# Autodesk Inventor assembly: skellett
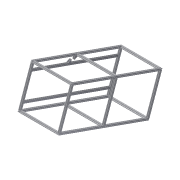
[picture p0: Inventor's stored thumbnail of the model, 180x180]
Saved by Autodesk Inventor 2014 SP1 (Build 180222100, 222)
## iProperties
Created: 2015-02-04
Part Number: skellett
Document SubType Name: Assembly
Designer: Simen
Author: Simen
## Documents named in this file (9)
- C:\Users\Simen\Documents\git\Eit\skjellet\skellett.iam
- C:\Users\Simen\Documents\git\Eit\skjellet\KHFS5_2020_1000.ipt
- C:\Users\Simen\Documents\git\Eit\skjellet\KHFS5_2020_486.ipt
- C:\Users\Simen\Documents\git\Eit\skjellet\KHFS5_2020_386.ipt
- C:\Users\Simen\Documents\git\Eit\skjellet\KHFS5_2020_381.ipt
- C:\Users\Simen\Documents\git\Eit\skjellet\KHFS5_2020_391.ipt
- C:\Users\Simen\Documents\git\Eit\skjellet\KHFS5_2020_960.ipt
- C:\Users\Simen\Documents\git\Eit\skjellet\KHFS5_2020_47.ipt
- C:\Users\Simen\Documents\git\Eit\skjellet\jorneFester.iam
## Components (26 placed, 2 different names)
1. KHFS5-2020-4000:12 — Mate:44, Flush:60, Flush:61, Flush:62, Flush:63, Mate:45, Mate:46, Mate:47, Flush:64, Flush:65, Flush:66, Flush:77, Flush:78, Mate:59
2. KHFS5-2020-4000:13 — Mate:36, Mate:37, Flush:45, Flush:46, Flush:47, Flush:48, Mate:39, Flush:56, Flush:57, Mate:52, Flush:71, Mate:62, Flush:81, Flush:82, Mate:67, Flush:88, Flush:89
3. KHFS5-2020-4000:14 — Mate:33, Mate:34, Mate:35, Flush:42, Flush:43, Flush:44, Flush:49, Flush:50, Flush:51, Mate:38, Mate:40, Mate:41, Flush:52, Flush:53, Flush:54, Flush:55, Flush:80, Mate:65, Flush:83, Mate:66, Flush:85, Flush:86, Flush:87
4. KHFS5-2020-4000:15 — Mate:43, Flush:58, Flush:59, Mate:53, Flush:73, Flush:75, Mate:56, Flush:76, Mate:58
5. KHFS5-2020-4000:25 — Mate:33, Flush:44, Flush:49
6. KHFS5-2020-4000:26 — Mate:34, Flush:43, Flush:51, Flush:67, Flush:68
7. KHFS5-2020-4000:27 — Mate:35, Flush:42, Flush:50, Flush:62, Flush:63, Mate:45
8. KHFS5-2020-4000:36 — Flush:69, Mate:50, Mate:55, Mate:58, Mate:63
9. KHFS5-2020-4000:28 — Mate:36, Flush:45, Flush:48, Flush:69, Mate:49, Flush:70
10. KHFS5-2020-4000:29 — Mate:37, Flush:46, Flush:47
11. KHFS5-2020-4000:30 — Mate:38, Mate:39, Flush:52, Flush:53, Flush:56, Flush:57
12. KHFS5-2020-4000:31 — Mate:40, Flush:54, Flush:68, Flush:72, Flush:84
13. KHFS5-2020-4000:32 — Mate:43, Flush:58, Flush:59, Mate:44, Flush:60, Flush:61
14. KHFS5-2020-4000:33 — Mate:41, Flush:55, Flush:87
15. KHFS5-2020-4000:34 — Mate:47, Flush:64, Flush:66
16. KHFS5-2020-4000:42 — Mate:62, Flush:81, Flush:82, Mate:63, Mate:64
17. KHFS5-2020-4000:43 — Mate:65, Flush:83, Flush:84
18. KHFS5-2020-4000:35 — Mate:46, Flush:65, Flush:67, Flush:74
19. KHFS5-2020-4000:37 — Mate:49, Flush:70, Mate:50, Mate:64
20. KHFS5-2020-4000:40 — Flush:77, Flush:78, Mate:59, Flush:80
21. KHFS5-2020-4000:38 — Mate:52, Flush:71, Flush:72
22. KHFS5-2020-4000:39 — Mate:53, Flush:73, Flush:74, Mate:54, Mate:57
23. jorneFester:1 [sub-assembly] — Mate:56, Mate:57, Flush:76
24. jorneFester:2 [sub-assembly] — Mate:54, Flush:75, Mate:55
25. KHFS5-2020-4000:44 — Mate:66, Flush:85, Flush:86
26. KHFS5-2020-4000:45 — Mate:67, Flush:88, Flush:89
## Relationships (78: Flush 47, Mate 31)
- Mate:33: KHFS5-2020-4000:14 ↔ KHFS5-2020-4000:25
- Mate:34: KHFS5-2020-4000:14 ↔ KHFS5-2020-4000:26
- Mate:35: KHFS5-2020-4000:14 ↔ KHFS5-2020-4000:27
- Mate:36: KHFS5-2020-4000:13 ↔ KHFS5-2020-4000:28
- Mate:37: KHFS5-2020-4000:13 ↔ KHFS5-2020-4000:29
- Flush:42: KHFS5-2020-4000:14 ↔ KHFS5-2020-4000:27
- Flush:43: KHFS5-2020-4000:14 ↔ KHFS5-2020-4000:26
- Flush:44: KHFS5-2020-4000:14 ↔ KHFS5-2020-4000:25
- Flush:45: KHFS5-2020-4000:13 ↔ KHFS5-2020-4000:28
- Flush:46: KHFS5-2020-4000:13 ↔ KHFS5-2020-4000:29
- Flush:47: KHFS5-2020-4000:13 ↔ KHFS5-2020-4000:29
- Flush:48: KHFS5-2020-4000:13 ↔ KHFS5-2020-4000:28
- Flush:49: KHFS5-2020-4000:14 ↔ KHFS5-2020-4000:25
- Flush:50: KHFS5-2020-4000:14 ↔ KHFS5-2020-4000:27
- Flush:51 (490 mm): KHFS5-2020-4000:14 ↔ KHFS5-2020-4000:26
- Mate:38: KHFS5-2020-4000:14 ↔ KHFS5-2020-4000:30
- Mate:39: KHFS5-2020-4000:13 ↔ KHFS5-2020-4000:30
- Mate:40: KHFS5-2020-4000:14 ↔ KHFS5-2020-4000:31
- Mate:41: KHFS5-2020-4000:14 ↔ KHFS5-2020-4000:33
- Flush:52: KHFS5-2020-4000:14 ↔ KHFS5-2020-4000:30
- Flush:53: KHFS5-2020-4000:14 ↔ KHFS5-2020-4000:30
- Flush:54: KHFS5-2020-4000:14 ↔ KHFS5-2020-4000:31
- Flush:55: KHFS5-2020-4000:14 ↔ KHFS5-2020-4000:33
- Flush:56: KHFS5-2020-4000:13 ↔ KHFS5-2020-4000:30
- Flush:57: KHFS5-2020-4000:13 ↔ KHFS5-2020-4000:30
- Mate:43: KHFS5-2020-4000:15 ↔ KHFS5-2020-4000:32
- Flush:58: KHFS5-2020-4000:15 ↔ KHFS5-2020-4000:32
- Flush:59: KHFS5-2020-4000:15 ↔ KHFS5-2020-4000:32
- Mate:44: KHFS5-2020-4000:12 ↔ KHFS5-2020-4000:32
- Flush:60: KHFS5-2020-4000:12 ↔ KHFS5-2020-4000:32
- Flush:61: KHFS5-2020-4000:12 ↔ KHFS5-2020-4000:32
- Flush:62: KHFS5-2020-4000:12 ↔ KHFS5-2020-4000:27
- Flush:63: KHFS5-2020-4000:12 ↔ KHFS5-2020-4000:27
- Mate:45: KHFS5-2020-4000:12 ↔ KHFS5-2020-4000:27
- Mate:46: KHFS5-2020-4000:12 ↔ KHFS5-2020-4000:35
- Mate:47: KHFS5-2020-4000:12 ↔ KHFS5-2020-4000:34
- Flush:64: KHFS5-2020-4000:12 ↔ KHFS5-2020-4000:34
- Flush:65: KHFS5-2020-4000:12 ↔ KHFS5-2020-4000:35
- Flush:66: KHFS5-2020-4000:12 ↔ KHFS5-2020-4000:34
- Flush:67: KHFS5-2020-4000:26 ↔ KHFS5-2020-4000:35
- Flush:68: KHFS5-2020-4000:26 ↔ KHFS5-2020-4000:31
- [Mate]: KHFS5-2020-4000:36 ↔ KHFS5-2020-4000:28
- Flush:69: KHFS5-2020-4000:36 ↔ KHFS5-2020-4000:28
- Mate:49: KHFS5-2020-4000:28 ↔ KHFS5-2020-4000:37
- Flush:70: KHFS5-2020-4000:28 ↔ KHFS5-2020-4000:37
- Mate:50 (241 mm): KHFS5-2020-4000:36 ↔ KHFS5-2020-4000:37
- Mate:52: KHFS5-2020-4000:13 ↔ KHFS5-2020-4000:38
- Flush:71: KHFS5-2020-4000:13 ↔ KHFS5-2020-4000:38
- Flush:72: KHFS5-2020-4000:31 ↔ KHFS5-2020-4000:38
- Mate:53: KHFS5-2020-4000:15 ↔ KHFS5-2020-4000:39
- Flush:73: KHFS5-2020-4000:15 ↔ KHFS5-2020-4000:39
- Flush:74: KHFS5-2020-4000:35 ↔ KHFS5-2020-4000:39
- Mate:54: KHFS5-2020-4000:39 ↔ jorneFester:2
- Flush:75: KHFS5-2020-4000:15 ↔ jorneFester:2
- Mate:55: KHFS5-2020-4000:36 ↔ jorneFester:2
- Mate:56: KHFS5-2020-4000:15 ↔ jorneFester:1
- Mate:57: KHFS5-2020-4000:39 ↔ jorneFester:1
- Flush:76: KHFS5-2020-4000:15 ↔ jorneFester:1
- Mate:58 (52.5 mm): KHFS5-2020-4000:15 ↔ KHFS5-2020-4000:36
- Flush:77: KHFS5-2020-4000:12 ↔ KHFS5-2020-4000:40
- Flush:78: KHFS5-2020-4000:12 ↔ KHFS5-2020-4000:40
- Mate:59: KHFS5-2020-4000:12 ↔ KHFS5-2020-4000:40
- Flush:80: KHFS5-2020-4000:14 ↔ KHFS5-2020-4000:40
- Mate:62: KHFS5-2020-4000:13 ↔ KHFS5-2020-4000:42
- Flush:81: KHFS5-2020-4000:13 ↔ KHFS5-2020-4000:42
- Flush:82: KHFS5-2020-4000:13 ↔ KHFS5-2020-4000:42
- Mate:63: KHFS5-2020-4000:36 ↔ KHFS5-2020-4000:42
- Mate:64: KHFS5-2020-4000:42 ↔ KHFS5-2020-4000:37
- Mate:65: KHFS5-2020-4000:14 ↔ KHFS5-2020-4000:43
- Flush:83: KHFS5-2020-4000:14 ↔ KHFS5-2020-4000:43
- Flush:84: KHFS5-2020-4000:31 ↔ KHFS5-2020-4000:43
- Mate:66: KHFS5-2020-4000:14 ↔ KHFS5-2020-4000:44
- Flush:85: KHFS5-2020-4000:14 ↔ KHFS5-2020-4000:44
- Flush:86: KHFS5-2020-4000:14 ↔ KHFS5-2020-4000:44
- Flush:87: KHFS5-2020-4000:14 ↔ KHFS5-2020-4000:33
- Mate:67: KHFS5-2020-4000:13 ↔ KHFS5-2020-4000:45
- Flush:88: KHFS5-2020-4000:13 ↔ KHFS5-2020-4000:45
- Flush:89: KHFS5-2020-4000:13 ↔ KHFS5-2020-4000:45
